# Autodesk Inventor assembly: Selection_Ramp 1
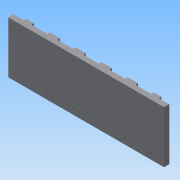
[picture p0: Inventor's stored thumbnail of the model, 180x180]
Saved by Autodesk Inventor 2018.1 (Build 221171000, 171)
## iProperties
Created: 2019-02-07
Part Number: Selection_Ramp 1
Document SubType Name: Assembly
Designer: James
Author: James
## Documents named in this file (4)
- C:\Users\admin\Desktop\Ball Sorting Machine\CAD\Selection_Ramp 1.iam
- C:\Users\admin\Desktop\Ball Sorting Machine\CAD\Selection_Ramp 1.ipt
- C:\Users\admin\Desktop\Ball Sorting Machine\CAD\Selection_Ramp 1_LHS Piece.ipt
- C:\Users\admin\Desktop\Ball Sorting Machine\CAD\Selection_Ramp 1_Mid piece.ipt
## Components (7 placed, 3 different names)
1. Selection_Ramp 1:1 — Flush:1, Flush:2, Flush:3, Mate:1, Mate:2, Mate:3, Flush:4, Flush:5, Mate:4, Flush:6, Flush:7, Mate:5, Mate:6, Mate:7, Mate:8, Mate:9, Flush:8, Flush:9
2. Selection_Ramp 1_LHS Piece:1 — Mate:7, Mate:8, Mate:9, Flush:8, Flush:9
3. Selection_Ramp 1_LHS Piece:2 — Mate:4, Flush:6, Flush:7, Mate:5, Mate:6
4. Selection_Ramp 1_Mid piece:1 — Mate:1, Mate:2, Mate:3, Flush:4, Flush:5
5. Selection_Ramp 1_Mid piece:2
6. Selection_Ramp 1_Mid piece:3
7. Selection_Ramp 1_Mid piece:4
## Component patterns: (4 elements, first: Selection_Ramp 1_Mid piece:1)
## Relationships (18: Flush 9, Mate 9)
- Flush:1: Selection_Ramp 1:1
- Flush:2: Selection_Ramp 1:1
- Flush:3: Selection_Ramp 1:1
- Mate:1: Selection_Ramp 1:1 ↔ Selection_Ramp 1_Mid piece:1
- Mate:2: Selection_Ramp 1:1 ↔ Selection_Ramp 1_Mid piece:1
- Mate:3: Selection_Ramp 1:1 ↔ Selection_Ramp 1_Mid piece:1
- Flush:4: Selection_Ramp 1:1 ↔ Selection_Ramp 1_Mid piece:1
- Flush:5: Selection_Ramp 1:1 ↔ Selection_Ramp 1_Mid piece:1
- Mate:4: Selection_Ramp 1:1 ↔ Selection_Ramp 1_LHS Piece:2
- Flush:6: Selection_Ramp 1:1 ↔ Selection_Ramp 1_LHS Piece:2
- Flush:7: Selection_Ramp 1:1 ↔ Selection_Ramp 1_LHS Piece:2
- Mate:5: Selection_Ramp 1:1 ↔ Selection_Ramp 1_LHS Piece:2
- Mate:6: Selection_Ramp 1:1 ↔ Selection_Ramp 1_LHS Piece:2
- Mate:7: Selection_Ramp 1:1 ↔ Selection_Ramp 1_LHS Piece:1
- Mate:8: Selection_Ramp 1:1 ↔ Selection_Ramp 1_LHS Piece:1
- Mate:9: Selection_Ramp 1:1 ↔ Selection_Ramp 1_LHS Piece:1
- Flush:8: Selection_Ramp 1:1 ↔ Selection_Ramp 1_LHS Piece:1
- Flush:9: Selection_Ramp 1:1 ↔ Selection_Ramp 1_LHS Piece:1
